# Autodesk Inventor assembly: dome_assembly
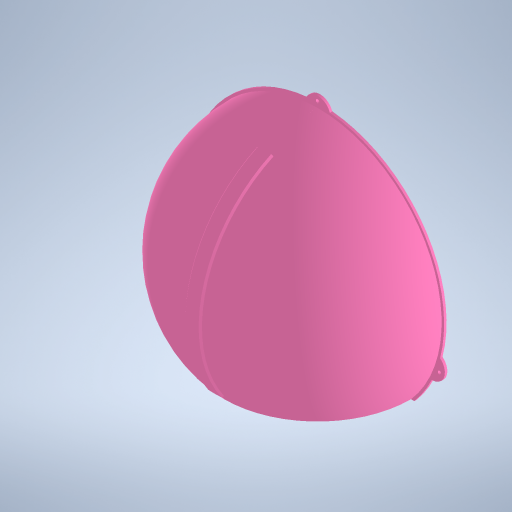
[picture p0: Inventor's stored thumbnail of the model, 512x512]
Saved by Autodesk Inventor 2024 (Build 280153000, 153)
## iProperties
Created: 2021-02-02
Part Number: dome_assembly
Document SubType Name: Assembly
Designer: dsdan
Author: dsdan
## Documents named in this file (4)
- E:\OneDrive - Imperial College London\DragonVision_DanielKo\Instrumentation\Ephys_rig_2021\Dome\dome_assembly.iam
- E:\OneDrive - Imperial College London\DragonVision_DanielKo\Instrumentation\Ephys_rig_2021\Dome\dome_mirror.ipt
- E:\OneDrive - Imperial College London\DragonVision_DanielKo\Instrumentation\Ephys_rig_2021\Dome\dome.ipt
- E:\OneDrive - Imperial College London\DragonVision_DanielKo\Instrumentation\Ephys_rig_2021\Dome\dummy.ipt
## Components (11 placed, 3 different names)
1. dome_mirror:1 — Mate:1, Mate:2, Flush:1, Mate:11, Mate:12, Mate:13
2. dome:1 — Mate:1, Mate:2, Flush:1, Flush:3
3. dummy:1 — Flush:3, Mate:13
4. dummy:2
5. dummy:3
6. dummy:4
7. dummy:5
8. dummy:6
9. dummy:7
10. dummy:8
11. dummy:9
## Component patterns: (9 elements, first: dummy:1)
## Relationships (8: Mate 5, Flush 3)
- Mate:1: dome_mirror:1 ↔ dome:1
- Mate:2: dome_mirror:1 ↔ dome:1
- Flush:1: dome_mirror:1 ↔ dome:1
- Flush:2 (198.5 mm)
- Flush:3: dome:1 ↔ dummy:1
- Mate:11: dome_mirror:1
- Mate:12: dome_mirror:1
- Mate:13: dome_mirror:1 ↔ dummy:1
